# Autodesk Inventor assembly: Assembly1
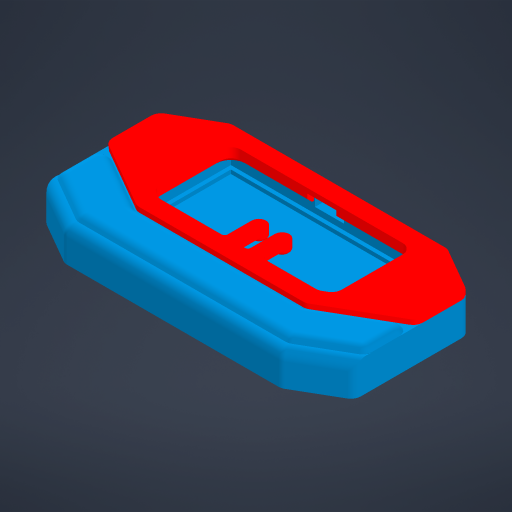
[picture p0: Inventor's stored thumbnail of the model, 512x512]
Saved by Autodesk Inventor 2023.4 (Build 274418000, 418)
## iProperties
Created: 2024-04-17
Part Number: Assembly1
Document SubType Name: Assembly
Designer: xSibe
Author: xSibe
## Documents named in this file (3)
- C:\.Laptop\.Work\Projects\Project Protocube\Protocube\CAD, STL, OBJ Files\1 CAD\Joystick\Gamepad Enclosure.iam
- C:\.Laptop\.Work\Projects\Project Protocube\Protocube\CAD, STL, OBJ Files\1 CAD\Joystick\Gamepad Bottom.ipt
- C:\.Laptop\.Work\Projects\Project Protocube\Protocube\CAD, STL, OBJ Files\1 CAD\Joystick\Gamepad Top.ipt
## Components (2 placed, 2 different names)
1. Gamepad Bottom:1 — Flush:1
2. Gamepad Top:1 — Flush:1
## Relationships (1: Flush 1)
- Flush:1: Gamepad Bottom:1 ↔ Gamepad Top:1
